# Autodesk Inventor assembly: LegoMan
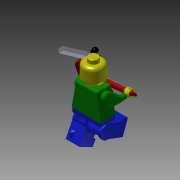
[picture p0: Inventor's stored thumbnail of the model, 180x180]
Saved by Autodesk Inventor 2015 (Build 190159000, 159)
## iProperties
Created: 2015-02-04
Part Number: LegoMan
Document SubType Name: Assembly
Designer: Paul
Author: Paul
## Documents named in this file (11)
- C:\Users\Paul\Google Drive\All #ResBaz Shared\Paul2AlizaCAD\06_Assembly\01_Lego_Man\LegoMan_GS_Answer.iam
- C:\Users\Paul\Google Drive\All #ResBaz Shared\Paul2AlizaCAD\06_Assembly\01_Lego_Man\TORSO.ipt
- C:\Users\Paul\Google Drive\All #ResBaz Shared\Paul2AlizaCAD\06_Assembly\01_Lego_Man\HIPS.ipt
- C:\Users\Paul\Google Drive\All #ResBaz Shared\Paul2AlizaCAD\06_Assembly\01_Lego_Man\LEG LHS.ipt
- C:\Users\Paul\Google Drive\All #ResBaz Shared\Paul2AlizaCAD\06_Assembly\01_Lego_Man\LEG RHS.ipt
- C:\Users\Paul\Google Drive\All #ResBaz Shared\Paul2AlizaCAD\06_Assembly\01_Lego_Man\ARM LHS.ipt
- C:\Users\Paul\Google Drive\All #ResBaz Shared\Paul2AlizaCAD\06_Assembly\01_Lego_Man\ARM RHS.ipt
- C:\Users\Paul\Google Drive\All #ResBaz Shared\Paul2AlizaCAD\06_Assembly\01_Lego_Man\HAND.ipt
- C:\Users\Paul\Google Drive\All #ResBaz Shared\Paul2AlizaCAD\06_Assembly\01_Lego_Man\HEAD.ipt
- C:\Users\Paul\Google Drive\All #ResBaz Shared\Paul2AlizaCAD\06_Assembly\01_Lego_Man\SWORD.ipt
- C:\Users\Paul\Google Drive\All #ResBaz Shared\Paul2AlizaCAD\06_Assembly\01_Lego_Man\GUITAR.ipt
## Components (11 placed, 10 different names)
1. TORSO:1 — Mate:1, Mate:2, Mate:3, Mate:8, Mate:9, Mate:10, Mate:11, Mate:16, Mate:17
2. HIPS:1 — Mate:1, Mate:2, Mate:3, Mate:4, Mate:5, Mate:6, Mate:7
3. LEG LHS:1 — Mate:4, Mate:5
4. LEG RHS:1 — Mate:6, Mate:7
5. ARM LHS:1 — Mate:8, Mate:9, Mate:12, Mate:13
6. ARM RHS:1 — Mate:10, Mate:11, Mate:14, Mate:15
7. HAND:1 — Mate:12, Mate:13, Mate:18, Mate:19
8. HAND:2 — Mate:14, Mate:15, Mate:20, Mate:21
9. HEAD:1 — Mate:16, Mate:17
10. GUITAR:1 — Mate:18, Mate:19
11. SWORD:1 — Mate:20, Mate:21
## Relationships (21: Mate 21)
- Mate:1: TORSO:1 ↔ HIPS:1
- Mate:2: TORSO:1 ↔ HIPS:1
- Mate:3: TORSO:1 ↔ HIPS:1
- Mate:4: HIPS:1 ↔ LEG LHS:1
- Mate:5: HIPS:1 ↔ LEG LHS:1
- Mate:6: HIPS:1 ↔ LEG RHS:1
- Mate:7: HIPS:1 ↔ LEG RHS:1
- Mate:8: TORSO:1 ↔ ARM LHS:1
- Mate:9: TORSO:1 ↔ ARM LHS:1
- Mate:10: TORSO:1 ↔ ARM RHS:1
- Mate:11: TORSO:1 ↔ ARM RHS:1
- Mate:12: ARM LHS:1 ↔ HAND:1
- Mate:13: ARM LHS:1 ↔ HAND:1
- Mate:14: ARM RHS:1 ↔ HAND:2
- Mate:15: ARM RHS:1 ↔ HAND:2
- Mate:16: TORSO:1 ↔ HEAD:1
- Mate:17: TORSO:1 ↔ HEAD:1
- Mate:18: HAND:1 ↔ GUITAR:1
- Mate:19: HAND:1 ↔ GUITAR:1
- Mate:20: HAND:2 ↔ SWORD:1
- Mate:21: HAND:2 ↔ SWORD:1
